# Autodesk Inventor assembly: RFID_and_holder
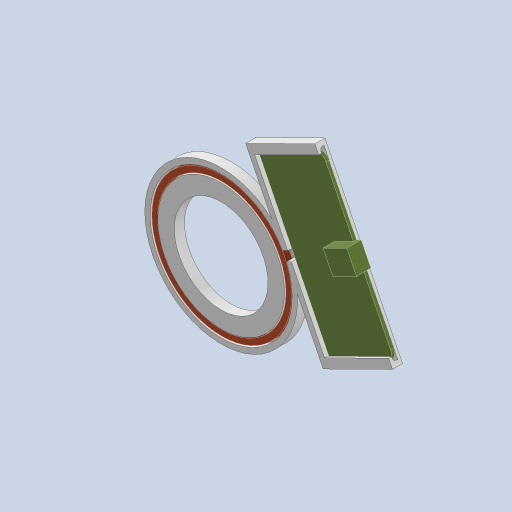
[picture p0: Inventor's stored thumbnail of the model, 512x512]
Saved by Autodesk Inventor 2024.4 (Build 284460000, 460)
## iProperties
Created: 2026-03-16
Part Number: RFID_and_holder
Document SubType Name: Assembly
Designer: tooles01
Author: tooles01
## Documents named in this file (4)
- C:\Users\tooles01\NYU Langone Health Dropbox\Shannon Toole\Shannon_Dropbox\Mar lab\RFID\CAD\RFID_and_holder.iam
- C:\Users\tooles01\NYU Langone Health Dropbox\Shannon Toole\Shannon_Dropbox\Mar lab\RFID\CAD\lib\RFID_coil.ipt
- C:\Users\tooles01\NYU Langone Health Dropbox\Shannon Toole\Shannon_Dropbox\Mar lab\RFID\CAD\lib\PCB.ipt
- C:\Users\tooles01\NYU Langone Health Dropbox\Shannon Toole\Shannon_Dropbox\Mar lab\RFID\CAD\RFID_holder_04.ipt
## Components (3 placed, 3 different names)
1. RFID_coil:1 — coil to holder
2. RFID_holder_04:1 — coil to holder, PCB base to holder base, PCB back to holder back, PCB to holder side
3. PCB:1 — PCB base to holder base, PCB back to holder back, PCB to holder side
## Relationships (4: Mate 3, Insert 1)
- coil to holder [Insert]: RFID_coil:1 ↔ RFID_holder_04:1
- PCB base to holder base [Mate]: RFID_holder_04:1 ↔ PCB:1
- PCB back to holder back [Mate]: RFID_holder_04:1 ↔ PCB:1
- PCB to holder side [Mate] (1 mm): RFID_holder_04:1 ↔ PCB:1
